# Autodesk Inventor assembly: FloorStingerTesting
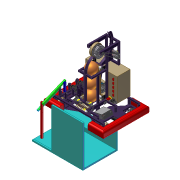
[picture p0: Inventor's stored thumbnail of the model, 180x180]
Saved by Autodesk Inventor 2012 (Build 160160000, 160)
## iProperties
Created: 2012-03-04
Part Number: FloorStingerTesting
Document SubType Name: Assembly
Designer: JesseK
Author: JesseK
## Documents named in this file (6)
- Z:\UserData\Documents\Inventor\team1885frc\Robot2012\FloorStingerTesting.iam
- Z:\UserData\Documents\Inventor\team1885frc\Bridge-FloorTester.ipt
- Z:\UserData\Documents\Inventor\team1885frc\Robot2012\RobotConceptTesting2.iam
- Z:\UserData\Documents\Inventor\team1885frc\Robot2012\BridgeLoweringDevice\Stinger.ipt
- Z:\UserData\Documents\Inventor\team1885frc\Robot2012\BridgeLoweringDevice\ExtensionTowerFor4-bar.ipt
- Z:\UserData\Documents\Inventor\team1885frc\Robot2012\BridgeLoweringDevice\StingerFoot.ipt
## Components (6 placed, 5 different names)
1. Bridge-FloorTester:1 — Flush:1, Flush:2, Mate:1
2. RobotConceptTesting2:1 [sub-assembly] — Flush:1, Flush:2, Mate:1, Flush:3, Mate:2, Flush:4, Flush:5, Mate:3
3. Stinger:1 — Flush:3, Mate:2, Mate:7
4. ExtensionTowerFor4-bar:1 — Flush:4, Flush:5, Mate:3, Mate:4, Mate:5
5. Stinger:2 — Mate:4, Mate:5, Flush:6, Mate:6
6. StingerFoot:1 — Flush:6, Mate:6, Mate:7
## Relationships (13: Mate 7, Flush 6)
- Flush:1: Bridge-FloorTester:1 ↔ RobotConceptTesting2:1
- Flush:2: Bridge-FloorTester:1 ↔ RobotConceptTesting2:1
- Mate:1 (88.9 mm): Bridge-FloorTester:1 ↔ RobotConceptTesting2:1
- Flush:3: RobotConceptTesting2:1 ↔ Stinger:1
- Mate:2: RobotConceptTesting2:1 ↔ Stinger:1
- Flush:4: RobotConceptTesting2:1 ↔ ExtensionTowerFor4-bar:1
- Flush:5: RobotConceptTesting2:1 ↔ ExtensionTowerFor4-bar:1
- Mate:3: RobotConceptTesting2:1 ↔ ExtensionTowerFor4-bar:1
- Mate:4: ExtensionTowerFor4-bar:1 ↔ Stinger:2
- Mate:5: ExtensionTowerFor4-bar:1 ↔ Stinger:2
- Flush:6: Stinger:2 ↔ StingerFoot:1
- Mate:6: Stinger:2 ↔ StingerFoot:1
- Mate:7: Stinger:1 ↔ StingerFoot:1
